# Autodesk Inventor assembly: BF6029
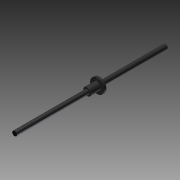
[picture p0: Inventor's stored thumbnail of the model, 180x180]
Saved by Autodesk Inventor 2011 (Build 150239000, 239)
## iProperties
Category: Miscellaneous
Company: Autodesk Inc.
Shininess: 64.0
Length Units: 11272
Angle Units: 11279
Time Units: 11290
Mass Units: 11286
Length Display Precision: 3
Angle Display Precision: 2
Compacted: True
Part Number: BF6029
Document SubType Name: Assembly
Created: 2008-01-12
Designer: Autodesk Inc.
Description: Lead Screw Assy
Vendor: Kerk Motion
Catalog Web Link: http://www.kerkmotion.com/products/lead-screw/b-series.asp
Density: 0.0
Volumn: 0.0
Area: 0.0
PropertySet Name: Model Information
Control State: 0
Master: False
Checked Out: False
Author: Autodesk Inc.
## Documents named in this file (3)
- R:\2012\Inventor\vkop\All_Miscellaneous\LeadScrew_KerkMotion_BF6029.iam
- R:\2012\Inventor\vkop\All_Miscellaneous\LeadScrew.ipt
- R:\2012\Inventor\vkop\All_Miscellaneous\LeadScrewNut.ipt
## Components (2 placed, 2 different names)
1. LeadScrew:1 — Mate:1
2. LeadScrewNut:1 — Mate:1
## Relationships (1: Mate 1)
- Mate:1: LeadScrew:1 ↔ LeadScrewNut:1
